# Autodesk Inventor assembly: lancerwheel
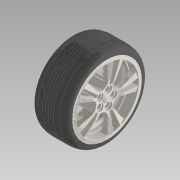
[picture p0: Inventor's stored thumbnail of the model, 180x180]
Saved by Autodesk Inventor 2021 (Build 250183000, 183)
## iProperties
Created: 2022-01-28
Part Number: lancerwheel
Document SubType Name: Assembly
Designer: juanc
Mass: 35317 g
Surface Area: 31087.7 cm^2
Volume: 16061.7 cm^3
Density: 2.19884 g/cm^3
Author: juanc
## Documents named in this file (3)
- H:\Mi unidad\2021 2\Robotica\Proyecto\modelado\griper\llanta\lancerwheel.iam
- H:\Mi unidad\2021 2\Robotica\Proyecto\modelado\griper\llanta\lancerrim.ipt
- H:\Mi unidad\2021 2\Robotica\Proyecto\modelado\griper\llanta\lancertire.ipt
## Components (2 placed, 2 different names)
1. lancerrim:1 — Mate:1, Mate:2
2. lancertire:1 — Mate:1, Mate:2
## Relationships (2: Mate 2)
- Mate:1: lancerrim:1 ↔ lancertire:1
- Mate:2: lancerrim:1 ↔ lancertire:1
